# Autodesk Inventor assembly: ShooterPrototype
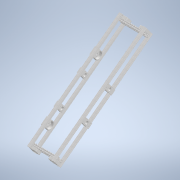
[picture p0: Inventor's stored thumbnail of the model, 180x180]
Saved by Autodesk Inventor 2020 (Build 240168000, 168)
## iProperties
Created: 2020-01-07
Part Number: ShooterPrototype
Document SubType Name: Assembly
Designer: srini
Author: srini
## Documents named in this file (6)
- C:\Users\srini\Documents\FRC\2020\ShooterPrototype.iam
- C:\Users\srini\Documents\FRC\2020\1003-48-CL.ipt
- C:\Users\srini\Documents\FRC\2020\9inSpacer.ipt
- C:\Users\srini\Documents\FRC\2020\1003-11-CL.ipt
- C:\Users\srini\Documents\FRC\2020\CIMmount.ipt
- C:\Users\srini\Documents\FRC\2020\BearingMount.ipt
## Components (18 placed, 5 different names)
1. 1003-48-CL:1 — Flush:1, Flush:2, Mate:1, Mate:2, Flush:3, Flush:4, Flush:8, Mate:3, Flush:9, Mate:4, Flush:11, Mate:27, Mate:28
2. 1003-48-CL:2 — Flush:1, Flush:2, Mate:1, Flush:7, Mate:5, Mate:6, Mate:23, Mate:24
3. 1003-48-CL:3 — Mate:2, Flush:3, Flush:4, Flush:5, Flush:6, Mate:7, Mate:10, Mate:13, Mate:19, Mate:20, Mate:21, Mate:22
4. 1003-48-CL:4 — Flush:5, Flush:6, Flush:7, Flush:10, Mate:8, Mate:9, Mate:14, Mate:17, Flush:16, Mate:18, Flush:17
5. 9inSpacer:1 — Flush:8, Flush:12, Flush:13, Flush:14, Flush:15, Mate:11, Mate:12
6. 9inSpacer:2 — Flush:10, Mate:7, Mate:8, Mate:15, Mate:16
7. 9inSpacer:3 — Mate:3, Flush:9, Mate:4
8. 9inSpacer:4 — Mate:5, Flush:11, Mate:6
9. 1003-11-CL:1 — Flush:12, Mate:9, Mate:12
10. 1003-11-CL:2 — Flush:13, Mate:10, Mate:11
11. 1003-11-CL:3 — Flush:14, Mate:14, Mate:15
12. 1003-11-CL:4 — Flush:15, Mate:13, Mate:16
13. CIMmount:1 — Mate:17, Flush:16, Flush:20
14. CIMmount:2 — Mate:18, Flush:17, Flush:18
15. BearingMount:1 — Mate:19, Mate:20, Mate:25, Flush:18, Flush:19
16. BearingMount:2 — Mate:21, Mate:22, Mate:26, Flush:19, Flush:20
17. BearingMount:3 — Mate:23, Mate:25, Mate:28
18. BearingMount:4 — Mate:24, Mate:26, Mate:27
## Relationships (48: Mate 28, Flush 20)
- Flush:1: 1003-48-CL:1 ↔ 1003-48-CL:2
- Flush:2: 1003-48-CL:1 ↔ 1003-48-CL:2
- Mate:1 (76.2 mm): 1003-48-CL:1 ↔ 1003-48-CL:2
- Mate:2 (228.6 mm): 1003-48-CL:1 ↔ 1003-48-CL:3
- Flush:3: 1003-48-CL:1 ↔ 1003-48-CL:3
- Flush:4: 1003-48-CL:1 ↔ 1003-48-CL:3
- Flush:5: 1003-48-CL:3 ↔ 1003-48-CL:4
- Flush:6: 1003-48-CL:3 ↔ 1003-48-CL:4
- Flush:7: 1003-48-CL:2 ↔ 1003-48-CL:4
- Flush:8: 1003-48-CL:1 ↔ 9inSpacer:1
- Mate:3: 1003-48-CL:1 ↔ 9inSpacer:3
- Flush:9: 1003-48-CL:1 ↔ 9inSpacer:3
- Mate:4: 1003-48-CL:1 ↔ 9inSpacer:3
- Flush:10: 1003-48-CL:4 ↔ 9inSpacer:2
- Mate:5: 1003-48-CL:2 ↔ 9inSpacer:4
- Flush:11: 1003-48-CL:1 ↔ 9inSpacer:4
- Mate:6: 1003-48-CL:2 ↔ 9inSpacer:4
- Mate:7: 1003-48-CL:3 ↔ 9inSpacer:2
- Mate:8: 1003-48-CL:4 ↔ 9inSpacer:2
- Flush:12: 9inSpacer:1 ↔ 1003-11-CL:1
- Flush:13: 9inSpacer:1 ↔ 1003-11-CL:2
- Flush:14: 9inSpacer:1 ↔ 1003-11-CL:3
- Flush:15: 9inSpacer:1 ↔ 1003-11-CL:4
- Mate:9: 1003-48-CL:4 ↔ 1003-11-CL:1
- Mate:10: 1003-48-CL:3 ↔ 1003-11-CL:2
- Mate:11: 9inSpacer:1 ↔ 1003-11-CL:2
- Mate:12: 9inSpacer:1 ↔ 1003-11-CL:1
- Mate:13: 1003-48-CL:3 ↔ 1003-11-CL:4
- Mate:14: 1003-48-CL:4 ↔ 1003-11-CL:3
- Mate:15: 9inSpacer:2 ↔ 1003-11-CL:3
- Mate:16: 9inSpacer:2 ↔ 1003-11-CL:4
- Mate:17: 1003-48-CL:4 ↔ CIMmount:1
- Flush:16: 1003-48-CL:4 ↔ CIMmount:1
- Mate:18: 1003-48-CL:4 ↔ CIMmount:2
- Flush:17: 1003-48-CL:4 ↔ CIMmount:2
- Mate:19: 1003-48-CL:3 ↔ BearingMount:1
- Mate:20: 1003-48-CL:3 ↔ BearingMount:1
- Mate:21: 1003-48-CL:3 ↔ BearingMount:2
- Mate:22: 1003-48-CL:3 ↔ BearingMount:2
- Mate:23: 1003-48-CL:2 ↔ BearingMount:3
- Mate:24: 1003-48-CL:2 ↔ BearingMount:4
- Mate:25: BearingMount:1 ↔ BearingMount:3
- Mate:26: BearingMount:2 ↔ BearingMount:4
- Mate:27: 1003-48-CL:1 ↔ BearingMount:4
- Mate:28: 1003-48-CL:1 ↔ BearingMount:3
- Flush:18 (167.325 mm): CIMmount:2 ↔ BearingMount:1
- Flush:19 (304.8 mm): BearingMount:1 ↔ BearingMount:2
- Flush:20 (167.325 mm): CIMmount:1 ↔ BearingMount:2
